# Autodesk Inventor assembly: Assembly1
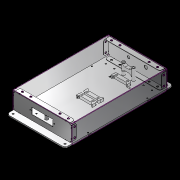
[picture p0: Inventor's stored thumbnail of the model, 180x180]
Saved by Autodesk Inventor 2018.2 (Build 222227000, 227)
## iProperties
Created: 2019-11-16
Part Number: Assembly1
Material: 一般
Document SubType Name: Assembly
Designer: gisen
Author: gisen
## Documents named in this file (7)
- C:\Users\gisen\Documents\CAD\inventor\ab_class_amp\Assembly1.iam
- C:\Users\gisen\Documents\CAD\inventor\ab_class_amp\bottom.ipt
- C:\Users\gisen\Documents\CAD\inventor\ab_class_amp\front.ipt
- C:\Users\gisen\Documents\CAD\inventor\ab_class_amp\dcdcfixer.ipt
- C:\Users\gisen\Documents\CAD\inventor\ab_class_amp\back.ipt
- C:\Users\gisen\Documents\CAD\inventor\ab_class_amp\top.ipt
- C:\Users\gisen\Documents\CAD\inventor\ab_class_amp\power_pcb_spacer_print.ipt
## Components (10 placed, 6 different names)
1. bottom:1 — メイト:1, メイト:2, メイト:3, メイト:4, メイト:5, メイト:6, メイト:7, メイト:8, メイト:9, メイト:10, メイト:11, メイト:12, メイト:13, メイト:14, メイト:15, メイト:16, メイト:17, メイト:18, メイト:21, メイト:22, メイト:23, メイト:24, メイト:25, メイト:26
2. front:1 — メイト:1, メイト:2, メイト:3, メイト:19, フラッシュ:1, メイト:20
3. dcdcfixer:1 — メイト:4, メイト:5, メイト:6
4. dcdcfixer:2 — メイト:7, メイト:8, メイト:9
5. dcdcfixer:3 — メイト:10, メイト:11, メイト:12
6. dcdcfixer:4 — メイト:13, メイト:14, メイト:15
7. back:1 — メイト:16, メイト:17, メイト:18
8. top:1 — メイト:19, フラッシュ:1, メイト:20
9. power_pcb_spacer_print:1 — メイト:21, メイト:24, メイト:25
10. power_pcb_spacer_print:2 — メイト:22, メイト:23, メイト:26
## Relationships (27: Mate 26, Flush 1)
- メイト:1 [Mate]: bottom:1 ↔ front:1
- メイト:2 [Mate]: bottom:1 ↔ front:1
- メイト:3 [Mate]: bottom:1 ↔ front:1
- メイト:4 [Mate]: bottom:1 ↔ dcdcfixer:1
- メイト:5 [Mate]: bottom:1 ↔ dcdcfixer:1
- メイト:6 [Mate]: bottom:1 ↔ dcdcfixer:1
- メイト:7 [Mate]: bottom:1 ↔ dcdcfixer:2
- メイト:8 [Mate]: bottom:1 ↔ dcdcfixer:2
- メイト:9 [Mate]: bottom:1 ↔ dcdcfixer:2
- メイト:10 [Mate]: bottom:1 ↔ dcdcfixer:3
- メイト:11 [Mate]: bottom:1 ↔ dcdcfixer:3
- メイト:12 [Mate]: bottom:1 ↔ dcdcfixer:3
- メイト:13 [Mate]: bottom:1 ↔ dcdcfixer:4
- メイト:14 [Mate]: bottom:1 ↔ dcdcfixer:4
- メイト:15 [Mate]: bottom:1 ↔ dcdcfixer:4
- メイト:16 [Mate]: bottom:1 ↔ back:1
- メイト:17 [Mate]: bottom:1 ↔ back:1
- メイト:18 [Mate]: bottom:1 ↔ back:1
- メイト:19 [Mate]: front:1 ↔ top:1
- フラッシュ:1 [Flush]: front:1 ↔ top:1
- メイト:20 [Mate]: front:1 ↔ top:1
- メイト:21 [Mate]: bottom:1 ↔ power_pcb_spacer_print:1
- メイト:22 [Mate]: bottom:1 ↔ power_pcb_spacer_print:2
- メイト:23 [Mate]: bottom:1 ↔ power_pcb_spacer_print:2
- メイト:24 [Mate]: bottom:1 ↔ power_pcb_spacer_print:1
- メイト:25 [Mate]: bottom:1 ↔ power_pcb_spacer_print:1
- メイト:26 [Mate]: bottom:1 ↔ power_pcb_spacer_print:2
